# Autodesk Inventor assembly: LargeSmallTransferGear
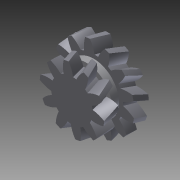
[picture p0: Inventor's stored thumbnail of the model, 180x180]
Saved by Autodesk Inventor 2012 (Build 160160000, 160)
## iProperties
Created: 2011-10-26
Part Number: LargeSmallTransferGear
Document SubType Name: Assembly
Designer: akutta
Author: akutta
## Documents named in this file (4)
- C:\Users\KuttaA\Dropbox\Hexapod Research\Leg Design\Other Parts\Intermediary Gear Box\Assemblies\LargeSmallTransferGear.iam
- C:\Users\KuttaA\Dropbox\Hexapod Research\Leg Design\Other Parts\Intermediary Gear Box\Assemblies\BlankGearLargeAndSmall.ipt
- C:\Users\KuttaA\Dropbox\Hexapod Research\Leg Design\Other Parts\Intermediary Gear Box\gear\Design Accelerator\Spur Gear11.ipt
- C:\Users\KuttaA\Dropbox\Hexapod Research\Leg Design\Other Parts\Intermediary Gear Box\gear\Design Accelerator\Spur Gear21.ipt
## Components (3 placed, 3 different names)
1. BlankGearLargeAndSmall:1 — Mate:1, Mate:2, Mate:3, Mate:4
2. Spur Gear1:1 — Mate:1, Mate:2
3. Spur Gear2:1 — Mate:3, Mate:4
## Relationships (4: Mate 4)
- Mate:1: BlankGearLargeAndSmall:1 ↔ Spur Gear1:1
- Mate:2: BlankGearLargeAndSmall:1 ↔ Spur Gear1:1
- Mate:3: BlankGearLargeAndSmall:1 ↔ Spur Gear2:1
- Mate:4: BlankGearLargeAndSmall:1 ↔ Spur Gear2:1
